# Autodesk Inventor assembly: gun
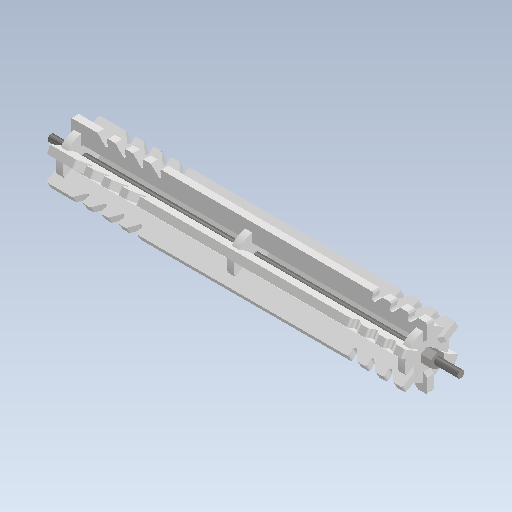
[picture p0: Inventor's stored thumbnail of the model, 512x512]
Saved by Autodesk Inventor 2020.1 (Build 241239000, 239)
## iProperties
Created: 2022-03-19
Part Number: gun
Document SubType Name: Assembly
Designer: User
Author: User
## Documents named in this file (5)
- D:\GitHub\TANK\3D-turret\gun.iam
- D:\GitHub\TANK\3D-turret\barrel_holder.ipt
- D:\GitHub\TANK\3D-turret\trunk.ipt
- D:\GitHub\TANK\3D-turret\ось пушки.ipt
- C:\Users\User\Documents\Inventor\Content Center Files\R2020\ru-RU\BS 4183(1)\BS 4183 - M4(1).ipt
## Components (16 placed, 4 different names)
1. barrel_holder:1 — Жесткий:7
2. barrel_holder:2 — Жесткий:1, Жесткий:2, Жесткий:3, Жесткий:4, Жесткий:5, Жесткий:6
3. trunk:1 — Жесткий:1, Жесткий:7
4. trunk:2 — Жесткий:2
5. trunk:3 — Жесткий:3
6. trunk:4 — Жесткий:4
7. trunk:5 — Жесткий:5
8. trunk:6 — Жесткий:6
9. BS 4183 - метрическая M4:1 — Жесткий:12
10. BS 4183 - метрическая M4:2 — Жесткий:13
11. BS 4183 - метрическая M4:3 — Жесткий:12, Жесткий:13
12. BS 4183 - метрическая M4:5 — Жесткий:15
13. BS 4183 - метрическая M4:6 — Жесткий:14
14. BS 4183 - метрическая M4:7 — Жесткий:14, Жесткий:15
15. ось пушки:1 — Жесткий:16
16. barrel_holder:3 — Жесткий:16
## Relationships (12: WeldJoint 12)
- Жесткий:1 [WeldJoint]: barrel_holder:2 ↔ trunk:1
- Жесткий:2 [WeldJoint]: barrel_holder:2 ↔ trunk:2
- Жесткий:3 [WeldJoint]: barrel_holder:2 ↔ trunk:3
- Жесткий:4 [WeldJoint]: barrel_holder:2 ↔ trunk:4
- Жесткий:5 [WeldJoint]: barrel_holder:2 ↔ trunk:5
- Жесткий:6 [WeldJoint]: barrel_holder:2 ↔ trunk:6
- Жесткий:7 [WeldJoint]: barrel_holder:1 ↔ trunk:1
- Жесткий:12 [WeldJoint]: BS 4183 - метрическая M4:1 ↔ BS 4183 - метрическая M4:3
- Жесткий:13 [WeldJoint]: BS 4183 - метрическая M4:2 ↔ BS 4183 - метрическая M4:3
- Жесткий:14 [WeldJoint]: BS 4183 - метрическая M4:6 ↔ BS 4183 - метрическая M4:7
- Жесткий:15 [WeldJoint]: BS 4183 - метрическая M4:5 ↔ BS 4183 - метрическая M4:7
- Жесткий:16 [WeldJoint]: ось пушки:1 ↔ barrel_holder:3
